# Autodesk Inventor assembly: mascon-new
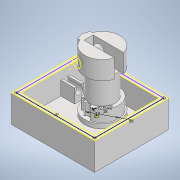
[picture p0: Inventor's stored thumbnail of the model, 180x180]
Saved by Autodesk Inventor 2021 (Build 250183000, 183)
## iProperties
Created: 2021-04-28
Part Number: mascon-new
Document SubType Name: Assembly
Designer: ben
Author: ben
## Documents named in this file (5)
- C:\Users\teh18\OneDrive\BVE Controller\r68-bve-mascon\mascon-new.iam
- C:\Users\teh18\OneDrive\BVE Controller\r68-bve-mascon\mascon.ipt
- C:\Users\teh18\OneDrive\BVE Controller\r68-bve-mascon\handle_base.ipt
- C:\Users\teh18\OneDrive\BVE Controller\r68-bve-mascon\handle_base2.ipt
- C:\Users\teh18\OneDrive\BVE Controller\r68-bve-mascon\stl2\HandleRod1.ipt
## Components (4 placed, 4 different names)
1. mascon:1
2. handle_base:1 — Flush:1, Flush:2
3. handle_base2:1 — Flush:1
4. HandleRod1:1 — Flush:2
## Relationships (2: Flush 2)
- Flush:1: handle_base:1 ↔ handle_base2:1
- Flush:2: handle_base:1 ↔ HandleRod1:1
